# Autodesk Inventor assembly: FINAL
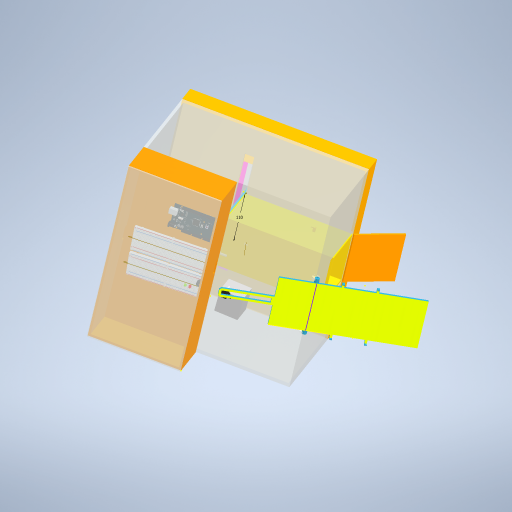
[picture p0: Inventor's stored thumbnail of the model, 512x512]
Saved by Autodesk Inventor 2024 (Build 280153000, 153)
## iProperties
Created: 2023-06-05
Part Number: FINAL
Document SubType Name: Assembly
Designer: hithi
Author: hithi
## Documents named in this file (18)
- C:\Users\hithi\OneDrive\Desktop\DS\FINAL.iam
- C:\Users\hithi\OneDrive\Desktop\DS\MAIN BODY.ipt
- C:\Users\hithi\OneDrive\Desktop\DS\bottom for door wheels.ipt
- C:\Users\hithi\OneDrive\Desktop\DS\CIRCUIT compartment.ipt
- C:\Users\hithi\OneDrive\Desktop\DS\ENTRY compartment.ipt
- C:\Users\hithi\Downloads\SPUR_06.ipt
- C:\Users\hithi\Downloads\RACK_06.ipt
- C:\Users\hithi\Downloads\Ultra Sonic Sensor\Ultra Sonic Sensor.ipt
- C:\Users\hithi\OneDrive\Desktop\Part422.ipt
- C:\Users\hithi\Downloads\buzzer-12x8-5mm-6-6m-pitch-1.snapshot.1\12085_buzzer\12085_buzzer\12085_buzzer.ipt
- C:\Users\hithi\Downloads\dm-s0020-2-1g-ultra-micro-servo-1.snapshot.2 (1)\DM-S0020 2.1G Ultra-Micro Servo v1\DM-S0020 2.1G Ultra-Micro Servo v1.ipt
- C:\Users\hithi\OneDrive\Desktop\DS\DSNDOOR 1.ipt
- C:\Users\hithi\Downloads\arduino_MEGA2650\arduino_MEGA2650.iam
- C:\Users\hithi\Downloads\Standard Large Breadboard with Two Side Rail\Standard Large Breadboard with Two Side Rail.iam
- C:\Users\hithi\Downloads\led-red-5mm-2.snapshot.1\BTG_901_BT_001_LED_5mm_Rot\LED_5mm_Rot.ipt
- C:\Users\hithi\Downloads\led-green-5mm-1.snapshot.1\BTG_901_BT_003_LED_5mm_Green\LED_5mm_Green.ipt
- C:\Users\hithi\OneDrive\Desktop\DS\wedge.ipt
- C:\Users\hithi\OneDrive\Desktop\abcd.ipt
## Components (20 placed, 17 different names)
1. MAIN BODY:1 — Mate:1, Mate:2, Mate:3, Mate:4, Mate:5, Mate:6, Mate:7, Mate:11, Mate:13, Mate:14, Mate:15, Mate:16, Mate:17, Mate:18, Mate:19, Mate:20
2. bottom for door wheels:1 — Mate:1, Mate:2, Mate:3, Mate:8, Mate:22, Mate:23
3. CIRCUIT compartment:1 — Mate:13, Mate:14, Mate:15, Mate:21, Mate:24, Mate:25, Mate:26
4. ENTRY compartment:1 — Mate:4, Mate:5, Mate:9, Mate:10, Mate:12
5. SPUR_06:1 — Mate:6, Mate:7
6. RACK_06:1 — Mate:8, Mate:9, Mate:10
7. Ultra Sonic Sensor:1 — Mate:12
8. Ultra Sonic Sensor:2 — Mate:11
9. Part422:1 — Mate:16, Mate:20
10. DM-S0020 2.1G Ultra-Micro Servo v1:1
11. DSNDOOR 1:1 — Mate:17, Mate:18, Mate:19
12. arduino_MEGA2650:1 [sub-assembly]
13. Standard Large Breadboard with Two Side Rail:1 [sub-assembly]
14. Standard Large Breadboard with Two Side Rail:2 [sub-assembly] — Mate:21
15. 12085_buzzer:1
16. LED_5mm_Rot:1
17. LED_5mm_Rot:2
18. LED_5mm_Green:1
19. wedge:1 — Mate:22, Mate:23
20. abcd:1 — Mate:24, Mate:25, Mate:26
## Relationships (26: Mate 26)
- Mate:1: MAIN BODY:1 ↔ bottom for door wheels:1
- Mate:2: MAIN BODY:1 ↔ bottom for door wheels:1
- Mate:3: MAIN BODY:1 ↔ bottom for door wheels:1
- Mate:4: MAIN BODY:1 ↔ ENTRY compartment:1
- Mate:5: MAIN BODY:1 ↔ ENTRY compartment:1
- Mate:6: MAIN BODY:1 ↔ SPUR_06:1
- Mate:7: MAIN BODY:1 ↔ SPUR_06:1
- Mate:8: bottom for door wheels:1 ↔ RACK_06:1
- Mate:9: ENTRY compartment:1 ↔ RACK_06:1
- Mate:10: ENTRY compartment:1 ↔ RACK_06:1
- Mate:11: MAIN BODY:1 ↔ Ultra Sonic Sensor:2
- Mate:12: ENTRY compartment:1 ↔ Ultra Sonic Sensor:1
- Mate:13: MAIN BODY:1 ↔ CIRCUIT compartment:1
- Mate:14: MAIN BODY:1 ↔ CIRCUIT compartment:1
- Mate:15: MAIN BODY:1 ↔ CIRCUIT compartment:1
- Mate:16: MAIN BODY:1 ↔ Part422:1
- Mate:17: MAIN BODY:1 ↔ DSNDOOR 1:1
- Mate:18: MAIN BODY:1 ↔ DSNDOOR 1:1
- Mate:19: MAIN BODY:1 ↔ DSNDOOR 1:1
- Mate:20: MAIN BODY:1 ↔ Part422:1
- Mate:21: CIRCUIT compartment:1 ↔ Standard Large Breadboard with Two Side Rail:2
- Mate:22: bottom for door wheels:1 ↔ wedge:1
- Mate:23: bottom for door wheels:1 ↔ wedge:1
- Mate:24: CIRCUIT compartment:1 ↔ abcd:1
- Mate:25: CIRCUIT compartment:1 ↔ abcd:1
- Mate:26: CIRCUIT compartment:1 ↔ abcd:1
